# Autodesk Inventor assembly: jezek_v_kleci
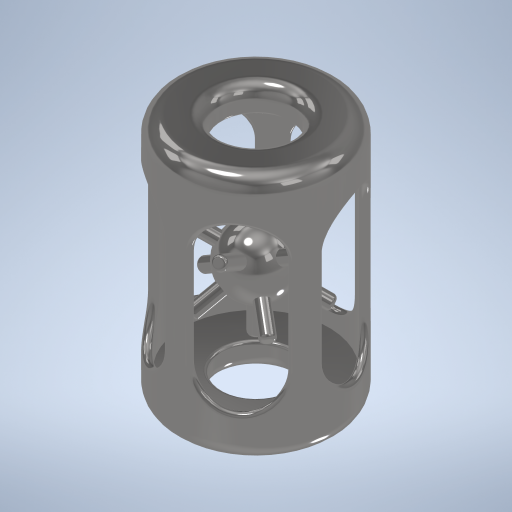
[picture p0: Inventor's stored thumbnail of the model, 512x512]
Saved by Autodesk Inventor 2023 (Build 270158000, 158)
## iProperties
Created: 2024-01-23
Part Number: jezek_v_kleci
Material: Všeobecné
Document SubType Name: Assembly
Designer: 42073
Mass: 34.3827 g
Surface Area: 183.79 cm^2
Volume: 34.3827 cm^3
Density: 1 g/cm^3
Author: 42073
## Documents named in this file (3)
- H:\mujgit\Skola\4L CAD\jezek_v_kleci.iam
- H:\mujgit\Skola\4L CAD\klec.ipt
- H:\mujgit\Skola\4L CAD\jezek v.ipt
## Components (2 placed, 2 different names)
1. klec:1 — Proti sobě:1, Stejný směr:1
2. jezek v:1 — Proti sobě:1, Stejný směr:1
## Relationships (2: Mate 1, Flush 1)
- Proti sobě:1 [Mate]: klec:1 ↔ jezek v:1
- Stejný směr:1 [Flush] (16.621 mm): klec:1 ↔ jezek v:1
